# Autodesk Inventor assembly: CornerWheel
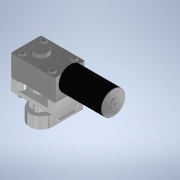
[picture p0: Inventor's stored thumbnail of the model, 180x180]
Saved by Autodesk Inventor 2020 (Build 240168000, 168)
## iProperties
Created: 2019-12-15
Part Number: CornerWheel
Document SubType Name: Assembly
Designer: Kjell
Mass: 435.462 g
Surface Area: 364.66 cm^2
Volume: 133.879 cm^3
Density: 3.25266 g/cm^3
Author: Kjell
## Documents named in this file (13)
- C:\Users\kjell\Documents\MarsRover\cad\CornerWheel.iam
- C:\Users\kjell\Documents\MarsRover\cad\ServoMount.ipt
- C:\Users\kjell\Documents\MarsRover\cad\ServoMotor.ipt
- C:\Users\kjell\Documents\MarsRover\cad\CornerWheel\Design Accelerator\Bearing1.iam
- C:\Users\kjell\Documents\MarsRover\cad\ServoShaft.ipt
- C:\Users\kjell\Documents\MarsRover\cad\ServoBBLid.ipt
- C:\Users\kjell\Documents\MarsRover\cad\CornerWheel\Design Accelerator\Bolted Connection3.iam
- C:\Users\kjell\Documents\MarsRover\cad\CornerWheel\Design Accelerator\Bolted Connection4.iam
- C:\Users\kjell\Documents\MarsRover\cad\CornerWheel\Design Accelerator\Bolted Connection5.iam
- C:\Users\kjell\Documents\MarsRover\cad\CornerWheel\Design Accelerator\Bolted Connection6.iam
- C:\Users\kjell\Documents\MarsRover\cad\CornerWheel\Design Accelerator\Bolted Connection7.iam
- C:\Users\kjell\Documents\MarsRover\cad\ServoArm.ipt
- C:\Users\kjell\Documents\MarsRover\cad\CornerWheel\Design Accelerator\Bolted Connection8.iam
## Components (13 placed, 7 different names)
1. ServoMount:1 — Rigid:2, Flush:1, Flush:2, Mate:3, Mate:5, Mate:7, Mate:9
2. ServoMotor:1 — Mate:4, Mate:6, Mate:8, Mate:10
3. Bearing:1 [sub-assembly] — Rigid:2, Rigid:3, Rotational:1
4. Bearing:2 [sub-assembly] — Rigid:3
5. ServoShaft:1 — Rotational:1, Flush:3, Flush:4
6. ServoBBLid:1 — Flush:1, Flush:2, Mate:1, Mate:2
7. Bolted Connection:1 [sub-assembly] — Mate:1, Mate:2
8. Bolted Connection:2 [sub-assembly] — Mate:3, Mate:4
9. Bolted Connection:3 [sub-assembly] — Mate:5, Mate:6
10. Bolted Connection:4 [sub-assembly] — Mate:7, Mate:8
11. Bolted Connection:5 [sub-assembly] — Mate:9, Mate:10
12. ServoArm:1 — Flush:3, Flush:4, Mate:11, Mate:12
13. Bolted Connection:6 [sub-assembly] — Mate:11, Mate:12
## Relationships (19: Mate 12, Flush 4, WeldJoint 2, RevoluteJoint 1)
- Rigid:2 [WeldJoint]: ServoMount:1 ↔ Bearing:1
- Rigid:3 [WeldJoint]: Bearing:1 ↔ Bearing:2
- Rotational:1 [RevoluteJoint]: Bearing:1 ↔ ServoShaft:1
- Flush:1: ServoMount:1 ↔ ServoBBLid:1
- Flush:2: ServoMount:1 ↔ ServoBBLid:1
- Mate:1: ServoBBLid:1 ↔ Bolted Connection:1
- Mate:2: ServoBBLid:1 ↔ Bolted Connection:1
- Mate:3: ServoMount:1 ↔ Bolted Connection:2
- Mate:4: ServoMotor:1 ↔ Bolted Connection:2
- Mate:5: ServoMount:1 ↔ Bolted Connection:3
- Mate:6: ServoMotor:1 ↔ Bolted Connection:3
- Mate:7: ServoMount:1 ↔ Bolted Connection:4
- Mate:8: ServoMotor:1 ↔ Bolted Connection:4
- Mate:9: ServoMount:1 ↔ Bolted Connection:5
- Mate:10: ServoMotor:1 ↔ Bolted Connection:5
- Flush:3: ServoShaft:1 ↔ ServoArm:1
- Flush:4: ServoShaft:1 ↔ ServoArm:1
- Mate:11: ServoArm:1 ↔ Bolted Connection:6
- Mate:12: ServoArm:1 ↔ Bolted Connection:6
